# Autodesk Inventor assembly: Eslabón2
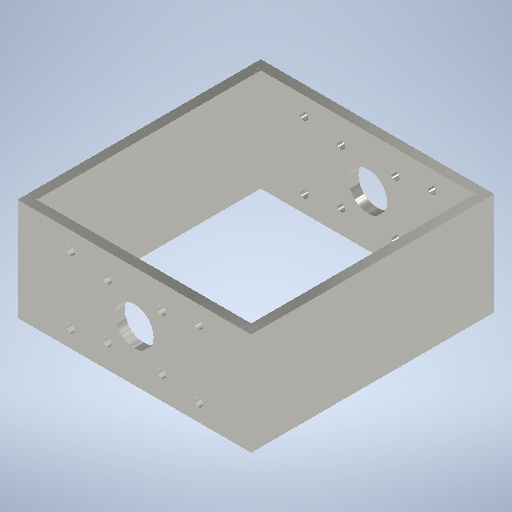
[picture p0: Inventor's stored thumbnail of the model, 512x512]
Saved by Autodesk Inventor 2025.1 (Build 291241000, 241)
## iProperties
Created: 2024-12-02
Part Number: Eslabón2
Document SubType Name: Assembly
Designer: Cristhian Vigo
Author: Cristhian Vigo
## Documents named in this file (3)
- D:\CRISTHIAN\universidad\ciclo 8\Robótica\PROYECTO\Modelo\ROBOT_5GDL\Eslabón2.iam
- D:\CRISTHIAN\universidad\ciclo 8\Robótica\PROYECTO\Modelo\ROBOT_5GDL\Base_eslabón.ipt
- D:\CRISTHIAN\universidad\ciclo 8\Robótica\PROYECTO\Modelo\ROBOT_5GDL\Eslabón2_Largo.ipt
## Components (3 placed, 2 different names)
1. Base_eslabón:1 — Flush:1, Flush:2, Mate:1
2. Eslabón2_Largo:1 — Flush:1, Flush:2, Mate:1, Flush:3, Flush:4, Mate:2
3. Base_eslabón:2 — Flush:3, Flush:4, Mate:2
## Relationships (6: Flush 4, Mate 2)
- Flush:1: Base_eslabón:1 ↔ Eslabón2_Largo:1
- Flush:2: Base_eslabón:1 ↔ Eslabón2_Largo:1
- Mate:1: Base_eslabón:1 ↔ Eslabón2_Largo:1
- Flush:3: Eslabón2_Largo:1 ↔ Base_eslabón:2
- Flush:4: Eslabón2_Largo:1 ↔ Base_eslabón:2
- Mate:2: Eslabón2_Largo:1 ↔ Base_eslabón:2
